# Autodesk Inventor assembly: Push
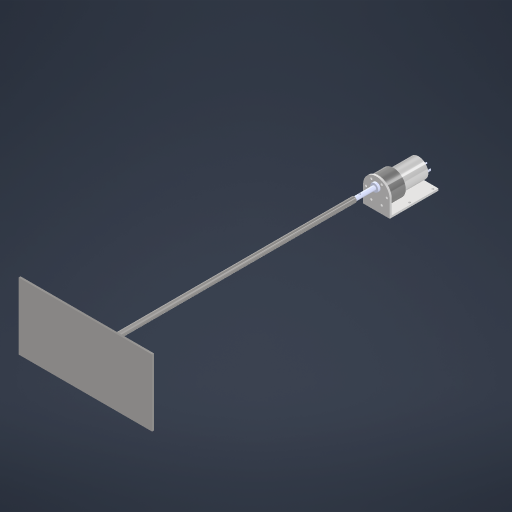
[picture p0: Inventor's stored thumbnail of the model, 512x512]
Saved by Autodesk Inventor 2023 (Build 270158000, 158)
## iProperties
Created: 2023-11-09
Part Number: Push
Document SubType Name: Assembly
Designer: Abhinav
Author: Abhinav
## Documents named in this file (4)
- C:\Users\Abhinav\Desktop\GRID\ARM 3\Orienter\Push.iam
- C:\Users\Abhinav\Desktop\GRID\ARM 3\Orienter\Push_motor_fix.ipt
- C:\Users\Abhinav\Desktop\GRID\ARM 3\Orienter\Screw.ipt
- C:\Users\Abhinav\Desktop\3D Library\Orange Motor.ipt
## Components (3 placed, 3 different names)
1. Push_motor_fix:1 — Mate:1, Mate:2, Mate:3, Angle:1
2. Screw:1 — Mate:4, Mate:5, Angle:1
3. Orange Motor:1 — Mate:1, Mate:2, Mate:3, Mate:4, Mate:5
## Relationships (6: Mate 5, Angle 1)
- Mate:1: Push_motor_fix:1 ↔ Orange Motor:1
- Mate:2: Push_motor_fix:1 ↔ Orange Motor:1
- Mate:3: Push_motor_fix:1 ↔ Orange Motor:1
- Mate:4: Screw:1 ↔ Orange Motor:1
- Mate:5: Screw:1 ↔ Orange Motor:1
- Angle:1 (0 deg): Push_motor_fix:1 ↔ Screw:1
